# Autodesk Inventor assembly: Cartesian2_YAssembly
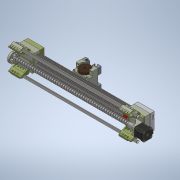
[picture p0: Inventor's stored thumbnail of the model, 180x180]
Saved by Autodesk Inventor 2020 (Build 240168000, 168)
## iProperties
Created: 2020-08-17
Part Number: Cartesian2_YAssembly
Material: Ogólny
Document SubType Name: Assembly
Designer: invin
Mass: 4227.11 g
Surface Area: 5602.37 cm^2
Volume: 1262.4 cm^3
Density: 3.34848 g/cm^3
Author: invin
## Documents named in this file (16)
- D:\KONIECTEGOKOŁCHOZU\MGR\Model\Workspaces\Obszar roboczy\assembly_v3\X\X.iam
- D:\KONIECTEGOKOŁCHOZU\MGR\Model\Workspaces\Obszar roboczy\content\item\item_0037003_Profile_5_20x20_L=564_1.ipt
- D:\KONIECTEGOKOŁCHOZU\MGR\Model\Workspaces\Obszar roboczy\content\manipulatorSharedParts\Cartesian1_12mm_Rod.ipt
- D:\KONIECTEGOKOŁCHOZU\MGR\Model\Workspaces\Obszar roboczy\content\manipulatorSharedParts\Cartesian2_BallBearing_25x37x7.ipt
- D:\KONIECTEGOKOŁCHOZU\MGR\Model\Workspaces\Obszar roboczy\Assembly_v1\X\OLD\Cartesian1_X_RodCover.ipt
- D:\KONIECTEGOKOŁCHOZU\MGR\Model\Workspaces\Obszar roboczy\content\nema17\Nema17 Stepper Motor.ipt
- D:\KONIECTEGOKOŁCHOZU\MGR\Model\Workspaces\Obszar roboczy\content\manipulatorSharedParts\Cartesian1_12_12_Clutch.ipt
- D:\KONIECTEGOKOŁCHOZU\MGR\Model\Workspaces\Obszar roboczy\content\manipulatorSharedParts\Cartesian1_BallScrew.ipt
- D:\KONIECTEGOKOŁCHOZU\MGR\Model\Workspaces\Obszar roboczy\content\igus\WJ200UM_01_10_1.ipt
- D:\KONIECTEGOKOŁCHOZU\MGR\Model\Workspaces\Obszar roboczy\assembly_v3\X\XSub1.iam
- D:\KONIECTEGOKOŁCHOZU\MGR\Model\Workspaces\Obszar roboczy\assembly_v3\X\XSub2.iam
- D:\KONIECTEGOKOŁCHOZU\MGR\Model\Workspaces\Obszar roboczy\assembly_v3\X\XItemEndCover.ipt
- D:\KONIECTEGOKOŁCHOZU\MGR\Model\Workspaces\Obszar roboczy\assembly_v3\X\XCarriage.ipt
- D:\KONIECTEGOKOŁCHOZU\MGR\Model\Workspaces\Obszar roboczy\assembly_v3\X\XCarriageNut.ipt
- D:\KONIECTEGOKOŁCHOZU\MGR\Model\Workspaces\Obszar roboczy\assembly_v3\X\XItemEnd.ipt
- D:\KONIECTEGOKOŁCHOZU\MGR\Model\Workspaces\Obszar roboczy\assembly_v3\X\XItemEndCoverConnector.ipt
## Components (23 placed, 15 different names)
1. XSub1:1 [sub-assembly] — Zestawiający:1, Kąt:1, Zestawiający:6, Zestawiający:7, Zestawiający:9, Zestawiający:10, Zestawiający:13, Zestawiający:32, Zestawiający:33, Zestawiający:34, Zestawiający:35, Zestawiający:36, Zestawiający:37, Zestawiający:44, Kąt:3, Zestawiający:45, Zestawiające:57, Zestawiające:75, Równoległe:14, Równoległe:15, Równoległe:17
2. XSub2:1 [sub-assembly] — Zestawiający:1, Kąt:1, Zestawiający:12, Równoległy:1, Równoległy:2, Zestawiający:24, Zestawiający:25, Zestawiający:26, Zestawiający:27, Zestawiający:28, Zestawiający:29, Zestawiający:30, Zestawiający:31, Zestawiające:50, Równoległe:3
3. XItemEnd:1 — Zestawiające:50, Zestawiające:52, Równoległe:3, Zestawiające:53, Równoległe:4, Równoległe:5, Zestawiające:55, Zestawiające:56
4. item_0037003_Profile_5_20x20_L=564_1:1 — Zestawiający:9, Zestawiający:10, Zestawiające:56, Równoległe:19
5. item_0037003_Profile_5_20x20_L=564_1:2 — Zestawiający:6, Zestawiający:7, Zestawiające:52, Zestawiające:55, Zestawiające:57, Zestawiające:58
6. Cartesian1_12mm_Rod:1 — Zestawiający:13, Równoległy:1
7. Cartesian1_12mm_Rod:2 — Zestawiający:12, Równoległy:2
8. Cartesian2_BallBearing_25x37x7:1 — Zestawiający:24, Zestawiający:25, Zestawiające:76
9. Cartesian1_X_RodCover:1 — Zestawiający:26, Zestawiający:27, Zestawiający:28
10. Cartesian1_X_RodCover:2 — Zestawiający:29, Zestawiający:30, Zestawiający:31
11. Cartesian1_X_RodCover:3 — Zestawiający:32, Zestawiający:33, Zestawiający:34
12. Cartesian1_X_RodCover:4 — Zestawiający:35, Zestawiający:36, Zestawiający:37
13. Nema17 Stepper Motor:2 — Zestawiający:44, Kąt:3, Zestawiający:45, Zestawiający:46, Zestawiający:47
14. Cartesian1_12_12_Clutch:1 — Zestawiający:46, Zestawiający:47, Zestawiający:48, Zestawiający:49
15. Cartesian1_BallScrew:1 — Zestawiający:48, Zestawiający:49
16. XItemEndCover:1 — Zestawiające:53, Równoległe:4, Równoległe:5, Równoległe:16
17. XCarriage:1 — Zestawiające:58, Zestawiające:59, Zestawiające:61, Zestawiające:62, Zestawiające:63, Zestawiające:64, Zestawiające:65, Zestawiające:66, Zestawiające:67, Zestawiające:68, Zestawiające:69, Zestawiające:70, Zestawiające:71, Zestawiające:72, Zestawiające:73, Równoległe:13, Równoległe:16, Zestawiające:77
18. XCarriageNut:1 — Zestawiające:59, Zestawiające:61
19. WJ200UM_01_10_1:1 — Zestawiające:62, Zestawiające:63, Zestawiające:64
20. WJ200UM_01_10_1:2 — Zestawiające:65, Zestawiające:66, Zestawiające:67
21. WJ200UM_01_10_1:3 — Zestawiające:68, Zestawiające:69, Zestawiające:70
22. WJ200UM_01_10_1:4 — Zestawiające:71, Zestawiające:72, Zestawiające:73
23. XItemEndCoverConnector:1 — Zestawiające:75, Równoległe:14, Równoległe:15
## Relationships (65: Mate 52, Flush 11, Angle 2)
- Zestawiający:1 [Mate]: XSub1:1 ↔ XSub2:1
- Kąt:1 [Angle] (0 deg): XSub1:1 ↔ XSub2:1
- Zestawiający:6 [Mate]: XSub1:1 ↔ item_0037003_Profile_5_20x20_L=564_1:2
- Zestawiający:7 [Mate]: XSub1:1 ↔ item_0037003_Profile_5_20x20_L=564_1:2
- Zestawiający:9 [Mate]: XSub1:1 ↔ item_0037003_Profile_5_20x20_L=564_1:1
- Zestawiający:10 [Mate]: XSub1:1 ↔ item_0037003_Profile_5_20x20_L=564_1:1
- Zestawiający:12 [Mate]: XSub2:1 ↔ Cartesian1_12mm_Rod:2
- Zestawiający:13 [Mate]: XSub1:1 ↔ Cartesian1_12mm_Rod:1
- Równoległy:1 [Flush] (4 mm): XSub2:1 ↔ Cartesian1_12mm_Rod:1
- Równoległy:2 [Flush] (4 mm): XSub2:1 ↔ Cartesian1_12mm_Rod:2
- Zestawiający:24 [Mate]: XSub2:1 ↔ Cartesian2_BallBearing_25x37x7:1
- Zestawiający:25 [Mate]: XSub2:1 ↔ Cartesian2_BallBearing_25x37x7:1
- Zestawiający:26 [Mate]: XSub2:1 ↔ Cartesian1_X_RodCover:1
- Zestawiający:27 [Mate]: XSub2:1 ↔ Cartesian1_X_RodCover:1
- Zestawiający:28 [Mate]: XSub2:1 ↔ Cartesian1_X_RodCover:1
- Zestawiający:29 [Mate]: XSub2:1 ↔ Cartesian1_X_RodCover:2
- Zestawiający:30 [Mate]: XSub2:1 ↔ Cartesian1_X_RodCover:2
- Zestawiający:31 [Mate]: XSub2:1 ↔ Cartesian1_X_RodCover:2
- Zestawiający:32 [Mate]: XSub1:1 ↔ Cartesian1_X_RodCover:3
- Zestawiający:33 [Mate]: XSub1:1 ↔ Cartesian1_X_RodCover:3
- Zestawiający:34 [Mate]: XSub1:1 ↔ Cartesian1_X_RodCover:3
- Zestawiający:35 [Mate]: XSub1:1 ↔ Cartesian1_X_RodCover:4
- Zestawiający:36 [Mate]: XSub1:1 ↔ Cartesian1_X_RodCover:4
- Zestawiający:37 [Mate]: XSub1:1 ↔ Cartesian1_X_RodCover:4
- Zestawiający:44 [Mate]: XSub1:1 ↔ Nema17 Stepper Motor:2
- Kąt:3 [Angle] (0 deg): XSub1:1 ↔ Nema17 Stepper Motor:2
- Zestawiający:45 [Mate]: XSub1:1 ↔ Nema17 Stepper Motor:2
- Zestawiający:46 [Mate]: Nema17 Stepper Motor:2 ↔ Cartesian1_12_12_Clutch:1
- Zestawiający:47 [Mate] (6 mm): Nema17 Stepper Motor:2 ↔ Cartesian1_12_12_Clutch:1
- Zestawiający:48 [Mate]: Cartesian1_12_12_Clutch:1 ↔ Cartesian1_BallScrew:1
- Zestawiający:49 [Mate]: Cartesian1_12_12_Clutch:1 ↔ Cartesian1_BallScrew:1
- Zestawiające:50 [Mate]: XSub2:1 ↔ XItemEnd:1
- Zestawiające:52 [Mate]: XItemEnd:1 ↔ item_0037003_Profile_5_20x20_L=564_1:2
- Równoległe:3 [Flush]: XSub2:1 ↔ XItemEnd:1
- Zestawiające:53 [Mate]: XItemEnd:1 ↔ XItemEndCover:1
- Równoległe:4 [Flush]: XItemEnd:1 ↔ XItemEndCover:1
- Równoległe:5 [Flush]: XItemEnd:1 ↔ XItemEndCover:1
- Zestawiające:55 [Mate]: XItemEnd:1 ↔ item_0037003_Profile_5_20x20_L=564_1:2
- Zestawiające:56 [Mate]: XItemEnd:1 ↔ item_0037003_Profile_5_20x20_L=564_1:1
- Zestawiające:57 [Mate]: XSub1:1 ↔ item_0037003_Profile_5_20x20_L=564_1:2
- Zestawiające:58 [Mate]: item_0037003_Profile_5_20x20_L=564_1:2 ↔ XCarriage:1
- Zestawiające:59 [Mate]: XCarriage:1 ↔ XCarriageNut:1
- Zestawiające:61 [Mate]: XCarriage:1 ↔ XCarriageNut:1
- Zestawiające:62 [Mate]: XCarriage:1 ↔ WJ200UM_01_10_1:1
- Zestawiające:63 [Mate]: XCarriage:1 ↔ WJ200UM_01_10_1:1
- Zestawiające:64 [Mate]: XCarriage:1 ↔ WJ200UM_01_10_1:1
- Zestawiające:65 [Mate]: XCarriage:1 ↔ WJ200UM_01_10_1:2
- Zestawiające:66 [Mate]: XCarriage:1 ↔ WJ200UM_01_10_1:2
- Zestawiające:67 [Mate]: XCarriage:1 ↔ WJ200UM_01_10_1:2
- Zestawiające:68 [Mate]: XCarriage:1 ↔ WJ200UM_01_10_1:3
- Zestawiające:69 [Mate]: XCarriage:1 ↔ WJ200UM_01_10_1:3
- Zestawiające:70 [Mate]: XCarriage:1 ↔ WJ200UM_01_10_1:3
- Zestawiające:71 [Mate]: XCarriage:1 ↔ WJ200UM_01_10_1:4
- Zestawiające:72 [Mate]: XCarriage:1 ↔ WJ200UM_01_10_1:4
- Zestawiające:73 [Mate]: XCarriage:1 ↔ WJ200UM_01_10_1:4
- Równoległe:13 [Flush]: XCarriage:1
- Zestawiające:75 [Mate]: XSub1:1 ↔ XItemEndCoverConnector:1
- Równoległe:14 [Flush]: XSub1:1 ↔ XItemEndCoverConnector:1
- Równoległe:15 [Flush]: XSub1:1 ↔ XItemEndCoverConnector:1
- Równoległe:16 [Flush] (-216 mm): XItemEndCover:1 ↔ XCarriage:1
- Równoległe:17 [Flush]: XSub1:1
- Zestawiające:76 [Mate]: Cartesian2_BallBearing_25x37x7:1
- Równoległe:19 [Flush] (-10 mm): item_0037003_Profile_5_20x20_L=564_1:1
- Zestawiające:77 [Mate]: XCarriage:1
- Zestawiające:78 [Mate]
